# Autodesk Inventor assembly: J008083
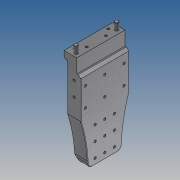
[picture p0: Inventor's stored thumbnail of the model, 180x180]
Saved by Autodesk Inventor 2018.3 (Build 223284000, 284)
## iProperties
RuleStatus: InUse
AfterDocSave0: file://Part Number Cleaner
Created: 2015-01-08
Vendor: HHMI: JFRC - ID&F
Document SubType Name: Assembly
Designer: ARNOLDJ
Mass: 370.391 g
Surface Area: 317.71 cm^2
Volume: 134.974 cm^3
Density: 2.74417 g/cm^3
Description: MBS OUTER POSARM NO GONIO
Project: COMMON
Part Number: J008083
ALTERED ITEM DESCRIPTION: N/A
ALTERED ITEM PART NUMBER: N/A
ALTERED ITEM VENDOR: N/A
DESIGN DEPARTMENT: HHMI: JRC - ID&F
LAB/DEPT: PACHITARIU (LAB)
REQUESTING SCIENTIST: PACHITARIU, MARIUS
SPECIAL FINISH: ANODIZE PER MIL-A-8625F, TYPE II, CLASS 2 (BLACK)
SURFACE ROUGHNESS: 63 Ra
Revision Number: -
## Documents named in this file (3)
- C:\_WORKSPACE\DATA\PROJECTS\_PROJECTS BY LAB\PACHITARIU (LAB)\BALL BEHAVIOR SETUP\MCAD\MBS OUTER POSARM NO GONIO.iam
- C:\_WORKSPACE\DATA\PROJECTS\_PROJECTS BY LAB\SVOBODA (LAB)\MOUSE POSITIONING SYSTEMS\MCAD\BALL SETUP\90145A512.ipt
- C:\_WORKSPACE\DATA\PROJECTS\_PROJECTS BY LAB\PACHITARIU (LAB)\BALL BEHAVIOR SETUP\MCAD\MBS OUTER POSARM NO GONIO.ipt
## Components (3 placed, 2 different names)
1. MBS OUTER POSARM NO GONIO:1 — Mate:6, Flush:4, Mate:7, Flush:5, Mate:8, Mate:9
2. 90145A512:1 — Mate:6, Flush:4
3. 90145A512:2 — Mate:7, Flush:5
## Relationships (8: Mate 5, Flush 3)
- Flush:3 (-59.3598 mm)
- Mate:6: MBS OUTER POSARM NO GONIO:1 ↔ 90145A512:1
- Flush:4 (-9.525 mm): MBS OUTER POSARM NO GONIO:1 ↔ 90145A512:1
- Mate:7: MBS OUTER POSARM NO GONIO:1 ↔ 90145A512:2
- Flush:5 (-9.525 mm): MBS OUTER POSARM NO GONIO:1 ↔ 90145A512:2
- Mate:8: MBS OUTER POSARM NO GONIO:1
- Mate:9: MBS OUTER POSARM NO GONIO:1
- Mate:10
